# Autodesk Inventor assembly: cutoutStator
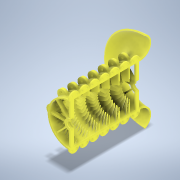
[picture p0: Inventor's stored thumbnail of the model, 180x180]
Saved by Autodesk Inventor 2021.2 (Build 252289000, 289)
## iProperties
Created: 2021-05-16
Part Number: cutoutStator
Document SubType Name: Assembly
Designer: Ryan
Author: Ryan
## Documents named in this file (8)
- C:\Users\Ryan\Documents\EDD\__NewCompressor\cutoutStator.iam
- C:\Users\Ryan\Documents\EDD\__NewCompressor\HalfShell.24.1.4.ipt
- C:\Users\Ryan\Documents\EDD\__NewCompressor\HalfShell.24.1.8.ipt
- C:\Users\Ryan\Documents\EDD\__NewCompressor\HalfShell.36.2.2.ipt
- C:\Users\Ryan\Documents\EDD\__NewCompressor\HalfShell.36.2.6.ipt
- C:\Users\Ryan\Documents\EDD\__NewCompressor\HalfShell.48.3.0.ipt
- C:\Users\Ryan\Documents\EDD\__NewCompressor\HalfShell.48.3.4.ipt
- C:\Users\Ryan\Documents\EDD\__NewCompressor\HalfInlet.ipt
## Components (7 placed, 7 different names)
1. HalfShell.24.1.4:1 — Insert:1, Insert:2
2. HalfShell.24.1.8:1 — Insert:2, Insert:3
3. HalfShell.36.2.2:1 — Insert:3, Insert:4
4. HalfShell.36.2.6:1 — Insert:4, Insert:5
5. HalfShell.48.3.0:1 — Insert:5, Insert:6
6. HalfShell.48.3.4:1 — Insert:6
7. HalfInlet:1 — Insert:1
## Relationships (6: Insert 6)
- Insert:1: HalfShell.24.1.4:1 ↔ HalfInlet:1
- Insert:2: HalfShell.24.1.4:1 ↔ HalfShell.24.1.8:1
- Insert:3: HalfShell.24.1.8:1 ↔ HalfShell.36.2.2:1
- Insert:4: HalfShell.36.2.2:1 ↔ HalfShell.36.2.6:1
- Insert:5: HalfShell.36.2.6:1 ↔ HalfShell.48.3.0:1
- Insert:6: HalfShell.48.3.0:1 ↔ HalfShell.48.3.4:1
